# Autodesk Inventor assembly: Series Elastic Gearbox
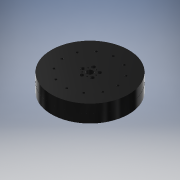
[picture p0: Inventor's stored thumbnail of the model, 180x180]
Saved by Autodesk Inventor 2017 SP1 (Build 210196100, 196)
## iProperties
Created: 2019-09-21
Part Number: Series Elastic Gearbox
Document SubType Name: Assembly
Designer: Dell
Author: Dell
## Documents named in this file (4)
- C:\Users\Zach\Documents\GitHub\tr2\Actuator 2.0\Series Elastic Gearbox 1.2\Series Elastic Gearbox 1.2.iam
- C:\Users\Zach\Documents\GitHub\tr2\Actuator 2.0\Series Elastic Gearbox 1.2\SG01.ipt
- C:\Users\Zach\Documents\GitHub\tr2\Actuator 2.0\Series Elastic Gearbox 1.2\SG02.ipt
- C:\Users\Zach\Documents\GitHub\tr2\Actuator 2.0\Series Elastic Gearbox 1.2\SG03.ipt
## Components (3 placed, 3 different names)
1. SG01:1 — Mate:1, Mate:2
2. SG02:1 — Mate:1, Mate:2, Mate:3, Mate:4
3. SG03:1 — Mate:3, Mate:4
## Relationships (4: Mate 4)
- Mate:1: SG01:1 ↔ SG02:1
- Mate:2: SG01:1 ↔ SG02:1
- Mate:3: SG02:1 ↔ SG03:1
- Mate:4: SG02:1 ↔ SG03:1
